# Autodesk Inventor assembly: Servomotor_1
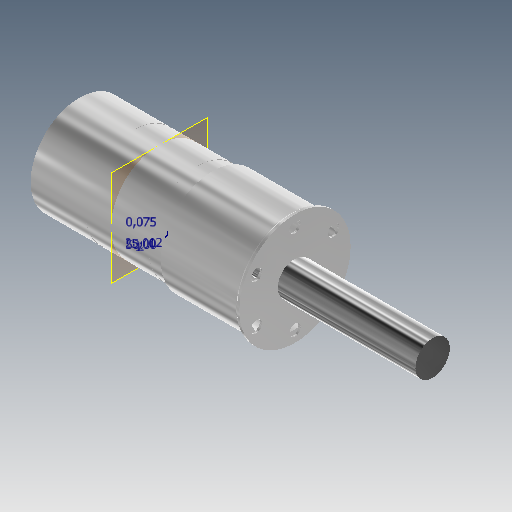
[picture p0: Inventor's stored thumbnail of the model, 512x512]
Saved by Autodesk Inventor 2020.3 (Build 243373010, 373A)
## iProperties
Created: 2021-04-09
Part Number: Servomotor_1
Document SubType Name: Assembly
Designer: marti
Mass: 209.98 g
Surface Area: 604.496 cm^2
Volume: 72.3614 cm^3
Density: 2.90182 g/cm^3
Author: marti
## Documents named in this file (10)
- C:\Users\marti\Documents\Inventor\RobotManipulateArm\17.4.2021 - Complete new IDEA\Servomotor_1.iam
- C:\Users\marti\Documents\Inventor\RobotManipulateArm\17.4.2021 - Complete new IDEA\Servo\Front cover of servo motor.ipt
- C:\Users\marti\Documents\Inventor\RobotManipulateArm\New parts\Cover for servomotor.ipt
- C:\Users\marti\Documents\Inventor\RobotManipulateArm\17.4.2021 - Complete new IDEA\Servo\PCB chip.iam
- C:\Users\marti\Documents\Inventor\RobotManipulateArm\17.4.2021 - Complete new IDEA\Servo\Flange motor side.ipt
- C:\Users\marti\Documents\Inventor\RobotManipulateArm\17.4.2021 - Complete new IDEA\Servo\Flange electronic side.ipt
- C:\Users\marti\Documents\Inventor\RobotManipulateArm\17.4.2021 - Complete new IDEA\Servo\Inner part of servo motor.ipt
- C:\Users\marti\Documents\Inventor\RobotManipulateArm\New parts\Back cover of servo motor.ipt
- C:\Users\marti\Documents\Inventor\RobotManipulateArm\17.4.2021 - Complete new IDEA\Servo\Thermal pad 2.ipt
- C:\Users\marti\Documents\Inventor\RobotManipulateArm\17.4.2021 - Complete new IDEA\Servo\Shaft1.ipt
## Components (9 placed, 9 different names)
1. Front cover of servo motor:1 — Mate:14, Mate:15, Mate:23
2. PCB chip:1 [sub-assembly] — Mate:3, Mate:4, Mate:5, Mate:16, Mate:17
3. Flange motor side:1 — Mate:6, Mate:7, Mate:8, Mate:9, Mate:11, Mate:12
4. Flange electronic side:1 — Mate:1, Mate:2, Mate:3, Mate:4, Mate:5, Mate:6, Mate:7, Mate:8, Flush:1
5. Inner part of servo motor:2 — Mate:9, Flush:1, Mate:10, Mate:13, Mate:18, Mate:19, Mate:20
6. Cover for servomotor:3 — Mate:11, Mate:12, Mate:13, Mate:14, Mate:15, Mate:21
7. Thermal pad 2:1 — Mate:17, Mate:18, Mate:19
8. Back cover of servo motor:1 — Mate:16, Mate:20, Mate:25
9. Shaft:1 — Mate:21, Mate:25
## Relationships (24: Mate 23, Flush 1)
- Mate:1: Flange electronic side:1
- Mate:2: Flange electronic side:1
- Mate:3: PCB chip:1 ↔ Flange electronic side:1
- Mate:4: PCB chip:1 ↔ Flange electronic side:1
- Mate:5: PCB chip:1 ↔ Flange electronic side:1
- Mate:6: Flange motor side:1 ↔ Flange electronic side:1
- Mate:7: Flange motor side:1 ↔ Flange electronic side:1
- Mate:8: Flange motor side:1 ↔ Flange electronic side:1
- Mate:9: Flange motor side:1 ↔ Inner part of servo motor:2
- Flush:1: Flange electronic side:1 ↔ Inner part of servo motor:2
- Mate:10: Inner part of servo motor:2
- Mate:11: Flange motor side:1 ↔ Cover for servomotor:3
- Mate:12: Flange motor side:1 ↔ Cover for servomotor:3
- Mate:13: Inner part of servo motor:2 ↔ Cover for servomotor:3
- Mate:14: Front cover of servo motor:1 ↔ Cover for servomotor:3
- Mate:15: Front cover of servo motor:1 ↔ Cover for servomotor:3
- Mate:16: PCB chip:1 ↔ Back cover of servo motor:1
- Mate:17: PCB chip:1 ↔ Thermal pad 2:1
- Mate:18: Inner part of servo motor:2 ↔ Thermal pad 2:1
- Mate:19: Inner part of servo motor:2 ↔ Thermal pad 2:1
- Mate:20: Inner part of servo motor:2 ↔ Back cover of servo motor:1
- Mate:21: Cover for servomotor:3 ↔ Shaft:1
- Mate:23: Front cover of servo motor:1
- Mate:25: Back cover of servo motor:1 ↔ Shaft:1
